# Autodesk Inventor assembly: звезда и втулка_MIR
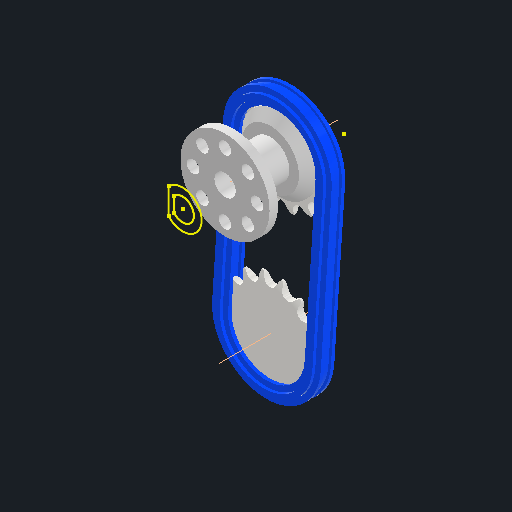
[picture p0: Inventor's stored thumbnail of the model, 512x512]
Saved by Autodesk Inventor 2025 (Build 290162000, 162)
## iProperties
Created: 2024-09-17
Part Number: звезда и втулка_MIR
Document SubType Name: Assembly
Designer: GameHD
Author: GameHD
## Documents named in this file (3)
- C:\Users\GameHD\Desktop\что-то нужное\Phantom16950\звезда и втулка_MIR.iam
- C:\Users\GameHD\Desktop\что-то нужное\Phantom16950\втулка для подш_MIR2.ipt
- C:\Users\GameHD\Desktop\что-то нужное\Phantom16950\цепь короткая 2.0_MIR1.ipt
## Components (2 placed, 2 different names)
1. втулка для подш_MIR2:1 — Заподлицо:1, Совмещение:1
2. цепь короткая 2.0_MIR1:1 — Заподлицо:1, Совмещение:1
## Relationships (2: Flush 1, Mate 1)
- Заподлицо:1 [Flush] (4 mm): втулка для подш_MIR2:1 ↔ цепь короткая 2.0_MIR1:1
- Совмещение:1 [Mate]: втулка для подш_MIR2:1 ↔ цепь короткая 2.0_MIR1:1
